# Autodesk Inventor assembly: HbIndexFingerForChild
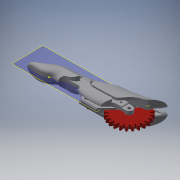
[picture p0: Inventor's stored thumbnail of the model, 180x180]
Saved by Autodesk Inventor 2018.1 (Build 221171000, 171)
## iProperties
Part Number: HbIndexFingerForChild
Material: 一般
Document SubType Name: Assembly
Designer: sktom
Author: sktom
## Documents named in this file (11)
- D:\CloudStrage\OneDrive\CAD\MAJ\hackberry\HACKberry-hardware\3D_69%inlength\Inventor\HbHandForChild\HbIndexFinger01ForChild\HbIndexFinger01ForChild.iam
- D:\CloudStrage\OneDrive\CAD\MAJ\hackberry\HACKberry-hardware\3D_69%inlength\Inventor\HbHandForChild\HbIndexFinger01ForChild\HbIndexMiddle-DistalPhalanx02ForChild.ipt
- D:\CloudStrage\OneDrive\CAD\MAJ\hackberry\HACKberry-hardware\3D_69%inlength\Inventor\HbHandForChild\HbIndexFinger01ForChild\HbIndexCouplerLink02ForChild.ipt
- D:\CloudStrage\OneDrive\CAD\MAJ\hackberry\HACKberry-hardware\3D_69%inlength\Inventor\HbHandForChild\HbIndexFinger01ForChild\HbIndexCouplerLinkCover02ForChild.ipt
- D:\CloudStrage\OneDrive\CAD\MAJ\hackberry\HACKberry-hardware\3D_69%inlength\Inventor\HbHandForChild\HbIndexFinger01ForChild\HbIndexProximalPhalanx03ForChild.ipt
- D:\CloudStrage\OneDrive\CAD\MAJ\hackberry\HACKberry-hardware\3D_69%inlength\Inventor\HbHandForChild\HbIndexFinger01ForChild\HbIndexProximalPhalanxCover02ForChild.ipt
- D:\CloudStrage\OneDrive\CAD\MAJ\hackberry\HACKberry-hardware\3D_69%inlength\Inventor\HbHandForChild\HbIndexFinger01ForChild\HbIndexReleaseLever02ForChild.ipt
- D:\CloudStrage\OneDrive\CAD\MAJ\hackberry\HACKberry-hardware\3D_69%inlength\Inventor\HbHandForChild\HbIndexFinger01ForChild\Spur Gear (24 teeth).ipt
- D:\CloudStrage\OneDrive\CAD\MAJ\hackberry\HACKberry-hardware\3D_69%inlength\Inventor\HbHandForChild\HbIndexFinger01ForChild\shaft_phi1.5_l6.ipt
- D:\CloudStrage\OneDrive\CAD\MAJ\hackberry\HACKberry-hardware\3D_69%inlength\Inventor\HbHandForChild\TOS 0.3-3-270ﾟ-3.ipt
- D:\CloudStrage\OneDrive\CAD\MAJ\hackberry\HACKberry-hardware\3D_69%inlength\Inventor\HbHandForChild\HbIndexFinger01ForChild\bolt_M1.4L6.ipt
## Components (16 placed, 10 different names)
1. HbIndexMiddle-DistalPhalanx02ForChild:1 — 円柱状:3, 挿入:17, 円柱状:4, 挿入:18, 挿入:20
2. HbIndexCouplerLink02ForChild:1 — 挿入:2, 挿入:3, 挿入:14
3. HbIndexCouplerLinkCover02ForChild:1 — 挿入:2, 挿入:3, 挿入:20, 挿入:21, 挿入:22
4. HbIndexProximalPhalanx03ForChild:1 — 挿入:15, 挿入:16, 挿入:23, 挿入:24
5. HbIndexProximalPhalanxCover02ForChild:1 — 円柱状:3, 挿入:15, 挿入:16, 挿入:18, 円柱状:5, 挿入:19, メイト:1
6. HbIndexReleaseLever02ForChild:1 — 回転:1, 挿入:19
7. Spur Gear (24 teeth):1 — 円柱状:5, メイト:1, 円柱状:6
8. shaft_phi1.5_l6:1 — 挿入:17, フラッシュ:1
9. shaft_phi1.5_l6:2 — 円柱状:4, フラッシュ:1
10. shaft_phi1.5_l6:3 — 回転:1
11. shaft_phi1.5_l6:4 — 挿入:14, 円柱状:6
12. TOS 0.3-3-270ﾟ-3:1
13. bolt_M1.4L6:1 — 挿入:21
14. bolt_M1.4L6:2 — 挿入:22
15. bolt_M1.4L6:3 — 挿入:23
16. bolt_M1.4L6:4 — 挿入:24
## Relationships (20: Insert 13, CylindricalJoint 4, Flush 1, RevoluteJoint 1, Mate 1)
- 挿入:2 [Insert]: HbIndexCouplerLink02ForChild:1 ↔ HbIndexCouplerLinkCover02ForChild:1
- 挿入:3 [Insert]: HbIndexCouplerLink02ForChild:1 ↔ HbIndexCouplerLinkCover02ForChild:1
- 挿入:14 [Insert] (-2 mm): HbIndexCouplerLink02ForChild:1 ↔ shaft_phi1.5_l6:4
- 円柱状:3 [CylindricalJoint]: HbIndexMiddle-DistalPhalanx02ForChild:1 ↔ HbIndexProximalPhalanxCover02ForChild:1
- 挿入:15 [Insert]: HbIndexProximalPhalanx03ForChild:1 ↔ HbIndexProximalPhalanxCover02ForChild:1
- 挿入:16 [Insert]: HbIndexProximalPhalanx03ForChild:1 ↔ HbIndexProximalPhalanxCover02ForChild:1
- 挿入:17 [Insert] (-0.8 mm): HbIndexMiddle-DistalPhalanx02ForChild:1 ↔ shaft_phi1.5_l6:1
- 円柱状:4 [CylindricalJoint]: HbIndexMiddle-DistalPhalanx02ForChild:1 ↔ shaft_phi1.5_l6:2
- フラッシュ:1 [Flush]: shaft_phi1.5_l6:1 ↔ shaft_phi1.5_l6:2
- 挿入:18 [Insert] (0.025 mm): HbIndexMiddle-DistalPhalanx02ForChild:1 ↔ HbIndexProximalPhalanxCover02ForChild:1
- 円柱状:5 [CylindricalJoint]: HbIndexProximalPhalanxCover02ForChild:1 ↔ Spur Gear (24 teeth):1
- 回転:1 [RevoluteJoint]: HbIndexReleaseLever02ForChild:1 ↔ shaft_phi1.5_l6:3
- 挿入:19 [Insert] (0.4 mm): HbIndexProximalPhalanxCover02ForChild:1 ↔ HbIndexReleaseLever02ForChild:1
- メイト:1 [Mate] (0.1 mm): HbIndexProximalPhalanxCover02ForChild:1 ↔ Spur Gear (24 teeth):1
- 円柱状:6 [CylindricalJoint]: Spur Gear (24 teeth):1 ↔ shaft_phi1.5_l6:4
- 挿入:20 [Insert] (0.1 mm): HbIndexMiddle-DistalPhalanx02ForChild:1 ↔ HbIndexCouplerLinkCover02ForChild:1
- 挿入:21 [Insert]: HbIndexCouplerLinkCover02ForChild:1 ↔ bolt_M1.4L6:1
- 挿入:22 [Insert]: HbIndexCouplerLinkCover02ForChild:1 ↔ bolt_M1.4L6:2
- 挿入:23 [Insert]: HbIndexProximalPhalanx03ForChild:1 ↔ bolt_M1.4L6:3
- 挿入:24 [Insert]: HbIndexProximalPhalanx03ForChild:1 ↔ bolt_M1.4L6:4
